# Autodesk Inventor assembly: Cup_Dispenser_Dynamic
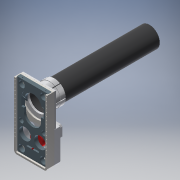
[picture p0: Inventor's stored thumbnail of the model, 180x180]
Saved by Autodesk Inventor 2016 (Build 200138000, 138)
## iProperties
Created: 2015-07-09
Part Number: Cup_Dispenser_Dynamic
Document SubType Name: Assembly
Designer: marku
Author: marku
## Documents named in this file (8)
- C:\Users\3DPrinterUser\Documents\GitHub\BarBot\Conception\Mechanical\Cup_Dispenser_Dynamic\Cup_Dispenser_Dynamic.iam
- C:\Users\3DPrinterUser\Documents\GitHub\BarBot\Conception\Mechanical\Cup_Dispenser_Dynamic\Cup_Dispenser_Hull.ipt
- C:\Users\3DPrinterUser\Documents\GitHub\BarBot\Conception\Mechanical\Cup_Dispenser_Dynamic\Cup_Dispenser_Fixture.ipt
- C:\Users\3DPrinterUser\Documents\GitHub\BarBot\Conception\Mechanical\Cup_Dispenser_Dynamic\Cup_Dispenser_Stepper_Montage.ipt
- C:\Users\3DPrinterUser\Documents\GitHub\BarBot\Conception\Mechanical\Cup_Dispenser_Dynamic\M1173041- NEMA 17.ipt
- C:\Users\3DPrinterUser\Documents\GitHub\BarBot\Conception\Mechanical\Cup_Dispenser_Dynamic\Cup_Dispenser_Slider.ipt
- C:\Users\3DPrinterUser\Documents\GitHub\BarBot\Conception\Mechanical\Cup_Dispenser_Dynamic\Cup_Dispenser_Transmission.ipt
- C:\Users\3DPrinterUser\Documents\GitHub\BarBot\Conception\Mechanical\Cup_Dispenser\Cup_Dispenser_Pipe.ipt
## Components (7 placed, 7 different names)
1. Cup_Dispenser_Hull:1 — Flush:1, Flush:2, Flush:3
2. Cup_Dispenser_Fixture:1 — Flush:1, Rotational:1
3. Cup_Dispenser_Stepper_Montage:1 — Flush:2, Rigid:1
4. M1173041- NEMA 17:1 — Rigid:1, Flush:5
5. Cup_Dispenser_Slider:1 — Flush:3, Flush:4
6. Cup_Dispenser_Transmission:1 — Flush:4, Flush:5
7. Cup_Dispenser_Pipe:1 — Rotational:1
## Relationships (7: Flush 5, WeldJoint 1, RevoluteJoint 1)
- Flush:1: Cup_Dispenser_Hull:1 ↔ Cup_Dispenser_Fixture:1
- Flush:2: Cup_Dispenser_Hull:1 ↔ Cup_Dispenser_Stepper_Montage:1
- Rigid:1 [WeldJoint]: Cup_Dispenser_Stepper_Montage:1 ↔ M1173041- NEMA 17:1
- Flush:3: Cup_Dispenser_Hull:1 ↔ Cup_Dispenser_Slider:1
- Flush:4: Cup_Dispenser_Slider:1 ↔ Cup_Dispenser_Transmission:1
- Flush:5: M1173041- NEMA 17:1 ↔ Cup_Dispenser_Transmission:1
- Rotational:1 [RevoluteJoint]: Cup_Dispenser_Fixture:1 ↔ Cup_Dispenser_Pipe:1
